# Autodesk Inventor assembly: Readout
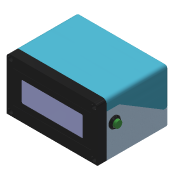
[picture p0: Inventor's stored thumbnail of the model, 180x180]
Saved by Autodesk Inventor 2020 (Build 240168000, 168)
## iProperties
Created: 2018-09-01
Part Number: Readout
Document SubType Name: Assembly
Designer: amsmi
Author: amsmi
## Documents named in this file (17)
- E:\My Documents\School\Pirani Supplemental Material\Low-Cost-Pirani-Gauge\3D Models (Inventor 2020)\Readout.iam
- E:\My Documents\School\Pirani Supplemental Material\Low-Cost-Pirani-Gauge\3D Models (Inventor 2020)\4x20 LCD.ipt
- E:\My Documents\School\Pirani Supplemental Material\Low-Cost-Pirani-Gauge\3D Models (Inventor 2020)\MicroUSB Breakout.iam
- E:\My Documents\School\Pirani Supplemental Material\Low-Cost-Pirani-Gauge\3D Models (Inventor 2020)\16 pin header.ipt
- E:\My Documents\School\Pirani Supplemental Material\Low-Cost-Pirani-Gauge\3D Models (Inventor 2020)\Gauge Controller.iam
- E:\My Documents\School\Pirani Supplemental Material\Low-Cost-Pirani-Gauge\3D Models (Inventor 2020)\PHS UNC19.ipt
- E:\My Documents\School\Pirani Supplemental Material\Low-Cost-Pirani-Gauge\3D Models (Inventor 2020)\PHS UNC20.ipt
- E:\My Documents\School\Pirani Supplemental Material\Low-Cost-Pirani-Gauge\3D Models (Inventor 2020)\PHS UNC2.ipt
- E:\My Documents\School\Pirani Supplemental Material\Low-Cost-Pirani-Gauge\3D Models (Inventor 2020)\Male Header - 1X2Wht.ipt
- E:\My Documents\School\Pirani Supplemental Material\Low-Cost-Pirani-Gauge\3D Models (Inventor 2020)\Switch Nut.ipt
- E:\My Documents\School\Pirani Supplemental Material\Low-Cost-Pirani-Gauge\3D Models (Inventor 2020)\Readout Wires.ipt
- E:\My Documents\School\Pirani Supplemental Material\Low-Cost-Pirani-Gauge\3D Models (Inventor 2020)\Readout Cover.ipt
- C:\Users\amsmi\Google Drive\Pirani Gauge\Pirani Gauge Modeling\Readout Rev 5\PHS UNC.ipt
- E:\My Documents\School\Pirani Supplemental Material\Low-Cost-Pirani-Gauge\3D Models (Inventor 2020)\Base2.ipt
- C:\Users\amsmi\Google Drive\Pirani Gauge\Pirani Gauge Modeling\Readout Rev 5\Male Headers.ipt
- E:\My Documents\School\Pirani Supplemental Material\Low-Cost-Pirani-Gauge\3D Models (Inventor 2020)\Clicker Switch.ipt
- E:\My Documents\School\Pirani Supplemental Material\Low-Cost-Pirani-Gauge\3D Models (Inventor 2020)\Faceplate.ipt
## Components (26 placed, 14 different names)
1. MicroUSB Breakout:1 [sub-assembly] — Flush:27, Mate:38, Flush:29, Insert:1, Insert:2, Flush:40, Flush:41, Flush:42
2. 16 pin header:1 — Mate:63, Mate:64, Mate:65
3. Gauge Controller:1 [sub-assembly] — Flush:27, Mate:38, Flush:29, Insert:3, Insert:4, Insert:5, Insert:6, Mate:48, Flush:34, Flush:35, Mate:49, Flush:36, Flush:37, Mate:58, Mate:59
4. Base2:1 — Mate:56, Mate:57, Mate:58, Mate:59, Mate:60, Flush:45, Flush:47
5. Clicker Switch:1 — Mate:56, Mate:57, Angle:1
6. PHS UNC19:1 — Insert:1
7. PHS UNC19:2 — Insert:2
8. PHS UNC19:3 — Insert:3
9. PHS UNC19:4 — Insert:5
10. PHS UNC19:5 — Insert:6
11. PHS UNC19:6 — Insert:4
12. PHS UNC20:7 — Insert:10
13. PHS UNC20:8 — Insert:9
14. PHS UNC2:9 — Insert:13
15. PHS UNC2:10 — Insert:12
16. PHS UNC2:12 — Insert:14
17. Male Header - 1X2Wht:1 — Mate:49, Flush:36, Flush:37, Mate:52, Mate:54, Flush:39
18. Male Header - 1X2Wht:2 — Mate:48, Flush:34, Flush:35
19. Switch Nut:1
20. Readout Wires:1 — Mate:52, Mate:54, Flush:39, Flush:40, Flush:41, Flush:42, Angle:1
21. Readout Cover:1
22. PHS UNC20:13 — Insert:7
23. PHS UNC20:14 — Insert:8
24. PHS UNC2:15 — Insert:11
25. Faceplate:1 — Mate:60, Flush:45, Flush:47, Flush:63, Insert:7, Insert:8, Insert:9, Insert:10, Flush:67, Flush:68
26. 4x20 LCD:4 — Flush:63, Insert:11, Insert:12, Insert:13, Insert:14, Mate:63, Mate:64, Mate:65, Flush:67, Flush:68
## Relationships (45: Flush 16, Mate 14, Insert 14, Angle 1)
- Flush:27: MicroUSB Breakout:1 ↔ Gauge Controller:1
- Mate:38 (3.175 mm): MicroUSB Breakout:1 ↔ Gauge Controller:1
- Flush:29: MicroUSB Breakout:1 ↔ Gauge Controller:1
- Insert:1: MicroUSB Breakout:1 ↔ PHS UNC19:1
- Insert:2: MicroUSB Breakout:1 ↔ PHS UNC19:2
- Insert:3: Gauge Controller:1 ↔ PHS UNC19:3
- Insert:4: Gauge Controller:1 ↔ PHS UNC19:6
- Insert:5: Gauge Controller:1 ↔ PHS UNC19:4
- Insert:6: Gauge Controller:1 ↔ PHS UNC19:5
- Mate:48: Gauge Controller:1 ↔ Male Header - 1X2Wht:2
- Flush:34: Gauge Controller:1 ↔ Male Header - 1X2Wht:2
- Flush:35: Gauge Controller:1 ↔ Male Header - 1X2Wht:2
- Mate:49: Gauge Controller:1 ↔ Male Header - 1X2Wht:1
- Flush:36: Gauge Controller:1 ↔ Male Header - 1X2Wht:1
- Flush:37: Gauge Controller:1 ↔ Male Header - 1X2Wht:1
- [Mate]: Base2:1 ↔ Switch Nut:1
- Mate:52: Male Header - 1X2Wht:1 ↔ Readout Wires:1
- Mate:54: Male Header - 1X2Wht:1 ↔ Readout Wires:1
- Flush:39: Male Header - 1X2Wht:1 ↔ Readout Wires:1
- Flush:40: MicroUSB Breakout:1 ↔ Readout Wires:1
- Flush:41: MicroUSB Breakout:1 ↔ Readout Wires:1
- Flush:42: MicroUSB Breakout:1 ↔ Readout Wires:1
- [Flush]: Base2:1 ↔ Readout Cover:1
- Mate:56: Base2:1 ↔ Clicker Switch:1
- Mate:57: Base2:1 ↔ Clicker Switch:1
- Angle:1 (180 deg): Clicker Switch:1 ↔ Readout Wires:1
- Mate:58: Gauge Controller:1 ↔ Base2:1
- Mate:59: Gauge Controller:1 ↔ Base2:1
- Mate:60: Base2:1 ↔ Faceplate:1
- Flush:45: Base2:1 ↔ Faceplate:1
- Flush:47: Base2:1 ↔ Faceplate:1
- Flush:63: Faceplate:1 ↔ 4x20 LCD:4
- Insert:7: PHS UNC20:13 ↔ Faceplate:1
- Insert:8: PHS UNC20:14 ↔ Faceplate:1
- Insert:9: PHS UNC20:8 ↔ Faceplate:1
- Insert:10: PHS UNC20:7 ↔ Faceplate:1
- Insert:11: PHS UNC2:15 ↔ 4x20 LCD:4
- Insert:12: PHS UNC2:10 ↔ 4x20 LCD:4
- Insert:13: PHS UNC2:9 ↔ 4x20 LCD:4
- Insert:14: PHS UNC2:12 ↔ 4x20 LCD:4
- Mate:63: 16 pin header:1 ↔ 4x20 LCD:4
- Mate:64: 16 pin header:1 ↔ 4x20 LCD:4
- Mate:65: 16 pin header:1 ↔ 4x20 LCD:4
- Flush:67: Faceplate:1 ↔ 4x20 LCD:4
- Flush:68: Faceplate:1 ↔ 4x20 LCD:4
